# Autodesk Inventor assembly: ASY МОО 020 конус
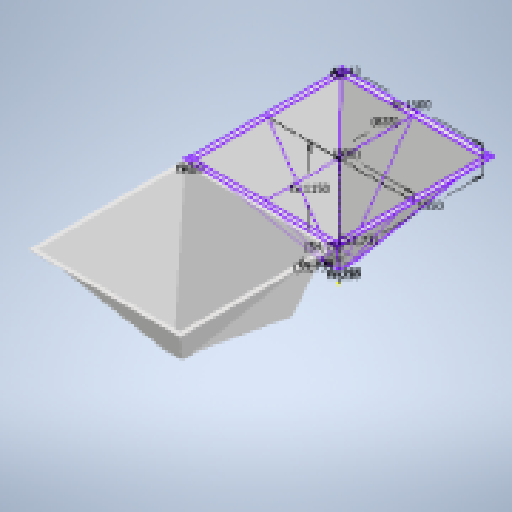
[picture p0: Inventor's stored thumbnail of the model, 512x512]
Saved by Autodesk Inventor 2024.2 (Build 282272000, 272)
## iProperties
Created: 2024-05-19
Part Number: ASY МОО 020 конус
Document SubType Name: Assembly
Designer: admin
Author: admin
## Documents named in this file (11)
- C:\Users\admin\YandexDisk-badmisterfox\домашниий пк\Inventor\Manturovo\Manturovo_Se-clar\ASY МОО 020 конус.iam
- C:\Users\admin\YandexDisk-badmisterfox\домашниий пк\Inventor\Manturovo\Manturovo_Se-clar\конус\МОО 023 конус подача правый борт.ipt
- C:\Users\admin\YandexDisk-badmisterfox\домашниий пк\Inventor\Manturovo\Manturovo_Se-clar\конус\МОО 029 конус подача дно.ipt
- C:\Users\admin\YandexDisk-badmisterfox\домашниий пк\Inventor\Manturovo\Manturovo_Se-clar\конус\МОО 025 конус подача левый борт.ipt
- C:\Users\admin\YandexDisk-badmisterfox\домашниий пк\Inventor\Manturovo\Manturovo_Se-clar\конус\МОО 022 конус подача корма.ipt
- C:\Users\admin\YandexDisk-badmisterfox\домашниий пк\Inventor\Manturovo\Manturovo_Se-clar\конус\МОО 021 конус эскиз .ipt
- C:\Users\admin\YandexDisk-badmisterfox\домашниий пк\Inventor\Manturovo\Manturovo_Se-clar\конус\МОО 026 конус подача нос.ipt
- C:\Users\admin\YandexDisk-badmisterfox\домашниий пк\Inventor\Manturovo\Manturovo_Se-clar\конус\МОО 032 конус выход корма.ipt
- C:\Users\admin\YandexDisk-badmisterfox\домашниий пк\Inventor\Manturovo\Manturovo_Se-clar\конус\МОО 030 конус выход правый борт.ipt
- C:\Users\admin\YandexDisk-badmisterfox\домашниий пк\Inventor\Manturovo\Manturovo_Se-clar\конус\МОО 031 конус выход левый борт.ipt
- C:\Users\admin\YandexDisk-badmisterfox\домашниий пк\Inventor\Manturovo\Manturovo_Se-clar\конус\МОО 033 конус выход нос.ipt
## Components (10 placed, 10 different names)
1. МОО 021 конус эскиз :1 — Flush:8, Flush:9, Mate:1
2. МОО 022 конус подача корма — Flush:6, Flush:10, Mate:2, Rigid:1, Rigid:2
3. МОО 029 конус подача дно:1 — Flush:4, Flush:5, Flush:11
4. МОО 023 конус подача правый борт:1 — Rigid:1, Rigid:3
5. МОО 025 конус подача левый борт:1 — Rigid:2
6. МОО 026 конус подача нос:1 — Rigid:3, Rigid:4
7. МОО 032 конус выход корма:1 — Rigid:4, Rigid:5, Rigid:6
8. МОО 030 конус выход правый борт:1 — Rigid:5, Rigid:7
9. МОО 031 конус выход левый борт:1 — Rigid:6
10. МОО 033 конус выход нос:1 — Rigid:7
## Relationships (16: Flush 7, WeldJoint 7, Mate 2)
- Flush:4: МОО 029 конус подача дно:1
- Flush:5: МОО 029 конус подача дно:1
- Flush:6: МОО 022 конус подача корма
- Flush:8: МОО 021 конус эскиз :1
- Flush:9: МОО 021 конус эскиз :1
- Mate:1: МОО 021 конус эскиз :1
- Flush:10: МОО 022 конус подача корма
- Mate:2: МОО 022 конус подача корма
- Flush:11 (-230 mm): МОО 029 конус подача дно:1
- Rigid:1 [WeldJoint]: МОО 022 конус подача корма ↔ МОО 023 конус подача правый борт:1
- Rigid:2 [WeldJoint]: МОО 022 конус подача корма ↔ МОО 025 конус подача левый борт:1
- Rigid:3 [WeldJoint]: МОО 023 конус подача правый борт:1 ↔ МОО 026 конус подача нос:1
- Rigid:4 [WeldJoint]: МОО 026 конус подача нос:1 ↔ МОО 032 конус выход корма:1
- Rigid:5 [WeldJoint]: МОО 032 конус выход корма:1 ↔ МОО 030 конус выход правый борт:1
- Rigid:6 [WeldJoint]: МОО 032 конус выход корма:1 ↔ МОО 031 конус выход левый борт:1
- Rigid:7 [WeldJoint]: МОО 030 конус выход правый борт:1 ↔ МОО 033 конус выход нос:1
